# Autodesk Inventor assembly: Belt Tensioner End_MIR
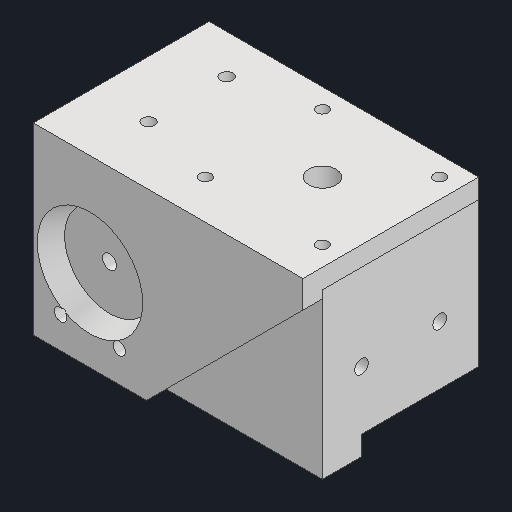
[picture p0: Inventor's stored thumbnail of the model, 512x512]
Saved by Autodesk Inventor 2025.1 (Build 291241000, 241)
## iProperties
Created: 2025-02-02
Part Number: Belt Tensioner End_MIR
Document SubType Name: Assembly
Designer: jerem
Author: jerem
## Documents named in this file (6)
- C:\Users\jerem\Documents\GitHub\Perovskite-Automated-Synthesis-System\CAD\Gantry\Belt Tensioner End_MIR.iam
- C:\Users\jerem\Documents\GitHub\Perovskite-Automated-Synthesis-System\CAD\Gantry\Idlert Tensioner_MIR.ipt
- C:\Users\jerem\Documents\GitHub\Perovskite-Automated-Synthesis-System\CAD\Gantry\tensionerholder_MIR.ipt
- C:\Users\jerem\Documents\GitHub\Perovskite-Automated-Synthesis-System\CAD\Gantry\X Axis End_MIR.ipt
- C:\Users\jerem\Documents\GitHub\Perovskite-Automated-Synthesis-System\CAD\Non 3D Printed Parts\Idler_MIR.ipt
- C:\Users\jerem\Documents\GitHub\Perovskite-Automated-Synthesis-System\CAD\Gantry\Tensioner Top_MIR.ipt
## Components (5 placed, 5 different names)
1. Idlert Tensioner_MIR:1 — Angle:2, Mate:2, Angle:1, Mate:4, Mate:3
2. tensionerholder_MIR:1 — Angle:2, Mate:2, Angle:1, Mate:1, Flush:2, Flush:1
3. X Axis End_MIR:1 — Mate:1, Flush:2, Flush:1, Mate:7, Mate:6, Mate:5
4. Idler_MIR:1 — Mate:4, Mate:3
5. Tensioner Top_MIR:1 — Mate:7, Mate:6, Mate:5
## Relationships (11: Mate 7, Angle 2, Flush 2)
- Angle:2 (0 deg): Idlert Tensioner_MIR:1 ↔ tensionerholder_MIR:1
- Mate:2: Idlert Tensioner_MIR:1 ↔ tensionerholder_MIR:1
- Angle:1 (180 deg): Idlert Tensioner_MIR:1 ↔ tensionerholder_MIR:1
- Mate:1: tensionerholder_MIR:1 ↔ X Axis End_MIR:1
- Flush:2: tensionerholder_MIR:1 ↔ X Axis End_MIR:1
- Flush:1: tensionerholder_MIR:1 ↔ X Axis End_MIR:1
- Mate:4: Idlert Tensioner_MIR:1 ↔ Idler_MIR:1
- Mate:3: Idlert Tensioner_MIR:1 ↔ Idler_MIR:1
- Mate:7: X Axis End_MIR:1 ↔ Tensioner Top_MIR:1
- Mate:6: X Axis End_MIR:1 ↔ Tensioner Top_MIR:1
- Mate:5: X Axis End_MIR:1 ↔ Tensioner Top_MIR:1
